# Autodesk Inventor assembly: Simulation_module
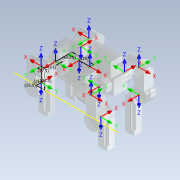
[picture p0: Inventor's stored thumbnail of the model, 180x180]
Saved by Autodesk Inventor 2020 (Build 240168000, 168)
## iProperties
Created: 2021-01-05
Part Number: Simulation_module
Document SubType Name: Assembly
Designer: DELL
Author: DELL
## Documents named in this file (5)
- F:\SoftRobot2.0\FlexipodHardware2.0\FlexipodHardware\Flexipod2.0\Cadquery_module\Simulation_module.iam
- F:\SoftRobot2.0\FlexipodHardware2.0\FlexipodHardware\Flexipod2.0\Cadquery_module\flexipod_body.ipt
- F:\SoftRobot2.0\FlexipodHardware2.0\FlexipodHardware\Flexipod2.0\Cadquery_module\flexipod_hip.ipt
- F:\SoftRobot2.0\FlexipodHardware2.0\FlexipodHardware\Flexipod2.0\Cadquery_module\flexipod_thigh.ipt
- F:\SoftRobot2.0\FlexipodHardware2.0\FlexipodHardware\Flexipod2.0\Cadquery_module\shank.ipt
## Components (13 placed, 4 different names)
1. flexipod_body:1 — Flush:4, Flush:1, Flush:5, Angle:1, Angle:2, Angle:3, Angle:4, Mate:1, Mate:2, Mate:3, Mate:4, Mate:5, Mate:6, Mate:7, Mate:8, Angle:5, Angle:6, Angle:7, Angle:8
2. flexipod_hip:1 — Angle:1, Mate:3, Mate:6, Mate:11, Mate:12
3. flexipod_hip:2 — Angle:2, Mate:4, Mate:5, Mate:9, Mate:10
4. flexipod_hip:3 — Angle:4, Mate:1, Mate:8, Mate:15, Mate:16
5. flexipod_hip:4 — Angle:3, Mate:2, Mate:7, Mate:13, Mate:14
6. flexipod_thigh:1 — Mate:11, Mate:12, Angle:6, Angle:12, Mate:18, Mate:25
7. flexipod_thigh:2 — Mate:9, Mate:10, Angle:5, Angle:11, Mate:19, Mate:24
8. flexipod_thigh:3 — Mate:13, Mate:14, Angle:7, Angle:9, Mate:20, Mate:22
9. flexipod_thigh:4 — Mate:15, Mate:16, Angle:8, Mate:17, Angle:10, Mate:21, Mate:23, Flush:6
10. shank:1 — Angle:12, Mate:18, Mate:25
11. shank:2 — Angle:11, Mate:19, Mate:24
12. shank:3 — Mate:17, Angle:10, Mate:21, Mate:23, Flush:7
13. shank:4 — Angle:9, Mate:20, Mate:22
## Relationships (42: Mate 25, Angle 12, Flush 5)
- Flush:4: flexipod_body:1
- Flush:1: flexipod_body:1
- Flush:5: flexipod_body:1
- Angle:1 (0 deg): flexipod_body:1 ↔ flexipod_hip:1
- Angle:2 (0 deg): flexipod_body:1 ↔ flexipod_hip:2
- Angle:3 (0 deg): flexipod_body:1 ↔ flexipod_hip:4
- Angle:4 (0 deg): flexipod_body:1 ↔ flexipod_hip:3
- Mate:1: flexipod_body:1 ↔ flexipod_hip:3
- Mate:2: flexipod_body:1 ↔ flexipod_hip:4
- Mate:3: flexipod_body:1 ↔ flexipod_hip:1
- Mate:4: flexipod_body:1 ↔ flexipod_hip:2
- Mate:5: flexipod_body:1 ↔ flexipod_hip:2
- Mate:6: flexipod_body:1 ↔ flexipod_hip:1
- Mate:7: flexipod_body:1 ↔ flexipod_hip:4
- Mate:8: flexipod_body:1 ↔ flexipod_hip:3
- Mate:9 (-10.5 mm): flexipod_hip:2 ↔ flexipod_thigh:2
- Mate:10: flexipod_hip:2 ↔ flexipod_thigh:2
- Angle:5 (0 deg): flexipod_body:1 ↔ flexipod_thigh:2
- Mate:11 (-10.5 mm): flexipod_hip:1 ↔ flexipod_thigh:1
- Mate:12: flexipod_hip:1 ↔ flexipod_thigh:1
- Angle:6 (0 deg): flexipod_body:1 ↔ flexipod_thigh:1
- Mate:13: flexipod_hip:4 ↔ flexipod_thigh:3
- Mate:14 (-10.5 mm): flexipod_hip:4 ↔ flexipod_thigh:3
- Angle:7 (0 deg): flexipod_body:1 ↔ flexipod_thigh:3
- Mate:15 (-10.5 mm): flexipod_hip:3 ↔ flexipod_thigh:4
- Mate:16: flexipod_hip:3 ↔ flexipod_thigh:4
- Angle:8 (0 deg): flexipod_body:1 ↔ flexipod_thigh:4
- Mate:17: flexipod_thigh:4 ↔ shank:3
- Angle:9 (0 deg): flexipod_thigh:3 ↔ shank:4
- Angle:10 (180 deg): flexipod_thigh:4 ↔ shank:3
- Angle:11 (0 deg): flexipod_thigh:2 ↔ shank:2
- Angle:12 (180 deg): flexipod_thigh:1 ↔ shank:1
- Mate:18: flexipod_thigh:1 ↔ shank:1
- Mate:19: flexipod_thigh:2 ↔ shank:2
- Mate:20: flexipod_thigh:3 ↔ shank:4
- Mate:21: flexipod_thigh:4 ↔ shank:3
- Mate:22: flexipod_thigh:3 ↔ shank:4
- Mate:23: flexipod_thigh:4 ↔ shank:3
- Mate:24: flexipod_thigh:2 ↔ shank:2
- Mate:25: flexipod_thigh:1 ↔ shank:1
- Flush:6: flexipod_thigh:4
- Flush:7: shank:3
